# Autodesk Inventor assembly: Suspenion_Arm_Assembly_V2
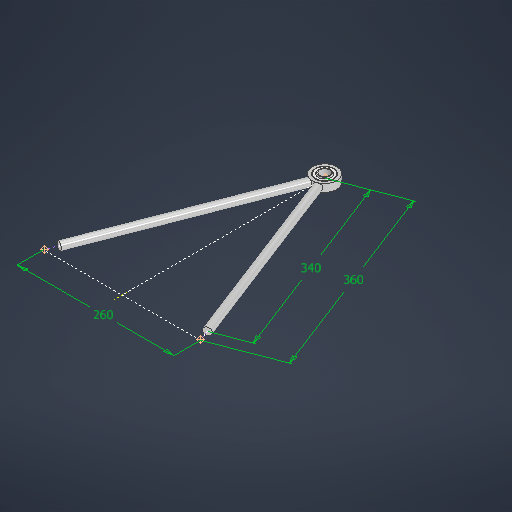
[picture p0: Inventor's stored thumbnail of the model, 512x512]
Saved by Autodesk Inventor 2026.1 (Build 301233000, 233)
## iProperties
_SolveAssemblyDoc: Frame Generator Solve Assembly
_Version: 15.0.0
Created: 2026-09-19
Part Number: Suspenion_Arm_Assembly_V2
Document SubType Name: Assembly
Designer: share
Author: share
## Documents named in this file (5)
- C:\Users\share\OneDrive\Documents\Personal Projects\GOGO Kart\CAD\GOGO_KART_FSAE\Suspension\Suspension_Arm_V2\Suspenion_Arm_Assembly_V2.iam
- C:\Users\share\OneDrive\Documents\Personal Projects\GOGO Kart\CAD\GOGO_KART_FSAE\Suspension\Suspension_Arm_V2\Suspenion_Arm_Outline_Sketch_V2.ipt
- C:\Users\share\OneDrive\Documents\Personal Projects\GOGO Kart\CAD\GOGO_KART_FSAE\Suspension\Suspension_Arm_V2\Outboard_Bearing_Housing.ipt
- C:\Users\share\OneDrive\Documents\Personal Projects\GOGO Kart\CAD\GOGO_KART_FSAE\Suspension\Suspension_Arm_V2\Suspenion_Arm_Assembly_V2\Frame\Frame 1789855613208.iam
- C:\Users\share\OneDrive\Documents\Personal Projects\GOGO Kart\CAD\GOGO_KART_FSAE\Suspension\Suspension_Arm_V2\63195K75_Swivel Joint (1).ipt
## Components (4 placed, 4 different names)
1. Suspenion_Arm_Outline_Sketch_V2:1 — Flush:1, Flush:2, Flush:3, Mate:3
2. Outboard_Bearing_Housing:1 — Mate:2, Mate:3, Mate:6
3. Frame 1789855613208:1 [sub-assembly]
4. 63195K75_Swivel Joint (1):1 — Mate:5, Mate:6
## Relationships (7: Mate 4, Flush 3)
- Flush:1: Suspenion_Arm_Outline_Sketch_V2:1
- Flush:2: Suspenion_Arm_Outline_Sketch_V2:1
- Flush:3: Suspenion_Arm_Outline_Sketch_V2:1
- Mate:2: Outboard_Bearing_Housing:1
- Mate:3: Suspenion_Arm_Outline_Sketch_V2:1 ↔ Outboard_Bearing_Housing:1
- Mate:5: 63195K75_Swivel Joint (1):1
- Mate:6: Outboard_Bearing_Housing:1 ↔ 63195K75_Swivel Joint (1):1
